# Autodesk Inventor assembly: shpon+podship
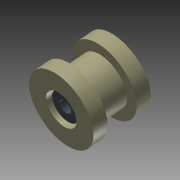
[picture p0: Inventor's stored thumbnail of the model, 180x180]
Saved by Autodesk Inventor 2015 (Build 190159000, 159)
## iProperties
Created: 2016-05-20
Part Number: shpon+podship
Document SubType Name: Assembly
Designer: Kostya
Author: Kostya
## Documents named in this file (3)
- C:\Users\criit\Documents\GitHub\LaserProject\ласт_ворк_v1.5.3\шпонька\shpon+podship.iam
- C:\Users\criit\Documents\GitHub\LaserProject\ласт_ворк_v1.5.3\шпонька\Katushka.ipt
- C:\Users\criit\Documents\GitHub\LaserProject\ласт_ворк_v1.5.3\шпонька\Podshipnik.ipt
## Components (3 placed, 2 different names)
1. Katushka:1 — Tangent:1, Tangent:2, Mate:1, Mate:2
2. Podshipnik:1 — Tangent:1, Mate:1
3. Podshipnik:2 — Tangent:2, Mate:2
## Relationships (4: Tangent 2, Mate 2)
- Tangent:1 (-2.5 mm): Katushka:1 ↔ Podshipnik:1
- Tangent:2 (-2.5 mm): Katushka:1 ↔ Podshipnik:2
- Mate:1: Katushka:1 ↔ Podshipnik:1
- Mate:2: Katushka:1 ↔ Podshipnik:2
